# Autodesk Inventor assembly: ABD_Version_0.1_leftleg
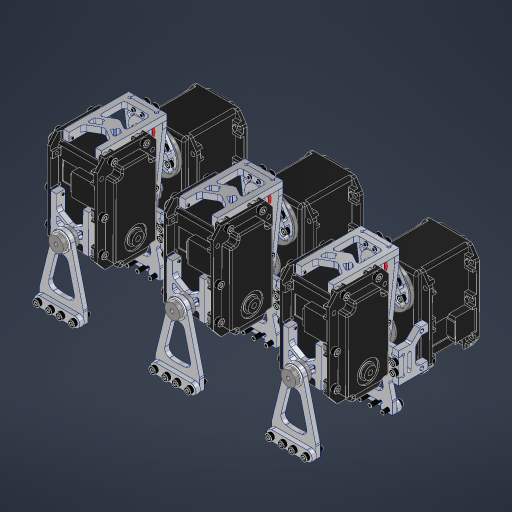
[picture p0: Inventor's stored thumbnail of the model, 512x512]
Saved by Autodesk Inventor 2024.3 (Build 283343000, 343)
## iProperties
Created: 2024-01-23
Part Number: ABD_Version_0.1_leftleg
Document SubType Name: Assembly
Designer: ASUS
Mass: 357.136 g
Surface Area: 604.848 cm^2
Volume: 181.423 cm^3
Density: 1.96853 g/cm^3
Author: ASUS
## Documents named in this file (26)
- C:\Users\ASUS\Desktop\Anti_Backlash_Structure_OP\v2_Frame\ABD_V2_Left_OP.iam
- C:\Users\ASUS\Desktop\ABD_2024_Eindhoven\MISUMI\Crank_Slider_Fixer.iam
- C:\Users\ASUS\Desktop\Anti_Backlash_Structure_OP\v2_Frame\Roll_Fixation_Set.iam
- C:\Users\ASUS\Desktop\Anti_Backlash_Structure_OP\v2_Frame\ABD_MX_64_Roll_Fixation_Set.iam
- C:\Users\ASUS\Desktop\Anti_Backlash_Structure_OP\v2_Frame\ABD_MX_64_Slider_Fixation_Set_Right2Horn.iam
- C:\Users\ASUS\Desktop\Anti_Backlash_Structure_OP\v2_Frame\ABD_Slider_Set_v2.iam
- C:\Users\ASUS\Desktop\Anti_Backlash_Structure_OP\v2_Frame\Roll_Fixation_Frame.ipt
- C:\Users\ASUS\Desktop\Anti_Backlash_Structure_OP\v2_Frame\Roll_Fixation_Frame_Back.ipt
- C:\Users\ASUS\Desktop\Anti_Backlash_Structure_OP\v2_Frame\hip joint fix washer.ipt
- C:\Users\ASUS\Desktop\ABD_2024_Eindhoven\MISUMI\hip_joint_fix_washer_10mm_Set.iam
- C:\Users\ASUS\Desktop\Anti_Backlash_Structure_OP\v2_Frame\Front_Frame_Fixer_v2.iam
- C:\Users\ASUS\Desktop\Anti_Backlash_Structure_OP\v2_Frame\Roll_Fixation_Frameto64.ipt
- C:\Users\ASUS\Desktop\ABD_2024_Eindhoven\MISUMI\CSH-ST-M2_5-6_203.ipt
- C:\Users\ASUS\Desktop\Anti_Backlash_Structure_OP\ROBOTIS(Inventor 2024 ver.)\DXL\MX-64T.ipt
- C:\Users\ASUS\Desktop\ABD_2024_Eindhoven\MISUMI\DBSY4-5-8.ipt
- C:\Users\ASUS\Desktop\ABD_2024_Eindhoven\MISUMI\C-WSSA12-4-2.ipt
- C:\Users\ASUS\Desktop\ABD_2024_Eindhoven\MISUMI\TT-0822-10.ipt
- C:\Users\ASUS\Desktop\ABD_2024_Eindhoven\MISUMI\CSHCS-SUSTBS-M4-20_214.ipt
- C:\Users\ASUS\Desktop\ABD_2024_Eindhoven\MISUMI\SLBNR4.ipt
- C:\Users\ASUS\Desktop\Anti_Backlash_Structure_OP\MISUMI\80F-0610.ipt
- C:\Users\ASUS\Desktop\ABD_2024_Eindhoven\MISUMI\C-WSSA12-8-3.ipt
- C:\Users\ASUS\Desktop\ABD_2024_Eindhoven\MISUMI\C-WSSA8-4-1.ipt
- C:\Users\ASUS\Desktop\Anti_Backlash_Structure_OP\V2_Frame(2025)\CSHBTT-ST-M4-18_203.ipt
- C:\Users\ASUS\Desktop\Anti_Backlash_Structure_OP\MISUMI\80F-0608.ipt
- C:\Users\ASUS\Desktop\ABD_2024_Eindhoven\MISUMI\E-GPWSSS12-4-1.ipt
- C:\Users\ASUS\Desktop\Anti_Backlash_Structure_OP\V2_Frame(2025)\M4-D6-9mm_Spacer.ipt
## Components (67 placed, 25 different names)
1. ABD_Slider_Set_v2:1 [sub-assembly]
2. Roll_Fixation_Set:1 [sub-assembly] — 삽입:5, 삽입:6, 각도:1, 플러쉬:4, 플러쉬:5, 플러쉬:7, 플러쉬:8, 메이트:43
3. Crank_Slider_Fixer:1 [sub-assembly] — 메이트:4
4. ABD_MX_64_Roll_Fixation_Set:1 [sub-assembly] — 메이트:2, 메이트:3, 삽입:5, 각도:1
5. ABD_MX_64_Slider_Fixation_Set_Right2Horn:1 [sub-assembly] — 메이트:2, 메이트:3, 삽입:6, 메이트:4
6. C-WSSA12-4-2:1 — 삽입:13, 삽입:15, 삽입:37
7. TT-0822-10:1 — 삽입:16, 삽입:36, 삽입:39
8. CSHCS-SUSTBS-M4-20_214:1
9. SLBNR4:1 — 삽입:13
10. 80F-0610:1 — 삽입:15, 삽입:16
11. Roll_Fixation_Frame:1
12. Roll_Fixation_Frame_Back:1 — 삽입:36
13. hip joint fix washer:1
14. hip joint fix washer:2
15. hip_joint_fix_washer_10mm_Set:1 [sub-assembly]
16. hip_joint_fix_washer_10mm_Set:2 [sub-assembly]
17. Front_Frame_Fixer_v2:1 [sub-assembly]
18. Roll_Fixation_Frameto64:1
19. Roll_Fixation_Frameto64:2
20. CSH-ST-M2_5-6_203:1
21. CSH-ST-M2_5-6_203:2
22. CSH-ST-M2_5-6_203:3
23. CSH-ST-M2_5-6_203:4
24. CSH-ST-M2_5-6_203:5
25. CSH-ST-M2_5-6_203:6
26. CSH-ST-M2_5-6_203:7
27. CSH-ST-M2_5-6_203:8
28. MX-64T:1 — 플러쉬:3, 메이트:26, 플러쉬:4, 플러쉬:5, 각도:2, 메이트:44
29. DBSY4-5-8:1
30. ABD_MX_64_Roll_Fixation_Set:2 [sub-assembly] — 삽입:37, 메이트:25, 각도:2
31. ABD_Slider_Set_v2:3 [sub-assembly] — 플러쉬:3, 메이트:26
32. Crank_Slider_Fixer:3 [sub-assembly]
33. ABD_MX_64_Slider_Fixation_Set_Right2Horn:3 [sub-assembly] — 삽입:39, 메이트:25, 삽입:40
34. C-WSSA12-8-3:1 — 삽입:40, 삽입:41
35. C-WSSA8-4-1:1 — 삽입:41, 삽입:42
36. CSHBTT-ST-M4-18_203:1 — 삽입:42
37. SLBNR4:2 — 삽입:83, 각도:4
38. Roll_Fixation_Frame:2
39. Roll_Fixation_Frame_Back:2 — 메이트:45
40. hip joint fix washer:3
41. hip joint fix washer:4
42. hip_joint_fix_washer_10mm_Set:3 [sub-assembly]
43. hip_joint_fix_washer_10mm_Set:4 [sub-assembly]
44. Front_Frame_Fixer_v2:2 [sub-assembly] — 삽입:85
45. Roll_Fixation_Frameto64:3
46. Roll_Fixation_Frameto64:4
47. CSH-ST-M2_5-6_203:9
48. CSH-ST-M2_5-6_203:10
49. CSH-ST-M2_5-6_203:11
50. CSH-ST-M2_5-6_203:12
51. CSH-ST-M2_5-6_203:13
52. CSH-ST-M2_5-6_203:14
53. CSH-ST-M2_5-6_203:15
54. CSH-ST-M2_5-6_203:16
55. MX-64T:2 — 플러쉬:7, 플러쉬:8, 메이트:43, 메이트:44
56. DBSY4-5-8:2
57. ABD_MX_64_Roll_Fixation_Set:3 [sub-assembly] — 삽입:82, 각도:4, 메이트:46, 삽입:85
58. ABD_Slider_Set_v2:4 [sub-assembly]
59. Crank_Slider_Fixer:4 [sub-assembly]
60. ABD_MX_64_Slider_Fixation_Set_Right2Horn:4 [sub-assembly] — 메이트:45, 메이트:46, 삽입:84
61. C-WSSA12-4-2:3 — 삽입:76, 삽입:82, 삽입:83
62. TT-0822-10:3 — 삽입:77, 삽입:78, 삽입:84
63. CSHBTT-ST-M4-18_203:3 — 삽입:79
64. 80F-0608:1 — 삽입:76, 삽입:77
65. TT-0822-10:4 — 삽입:78, 삽입:80
66. E-GPWSSS12-4-1:1 — 삽입:79, 삽입:81
67. M4-D6-9mm_Spacer:1 — 삽입:80, 삽입:81
## Relationships (111: Insert 63, Mate 38, Flush 6, Angle 4)
- [Insert]: ABD_Slider_Set_v2:1 ↔ Roll_Fixation_Set:1
- [Insert]: ABD_Slider_Set_v2:1 ↔ Crank_Slider_Fixer:1
- 메이트:2 [Mate] (0.05 mm): ABD_MX_64_Roll_Fixation_Set:1 ↔ ABD_MX_64_Slider_Fixation_Set_Right2Horn:1
- 메이트:3 [Mate]: ABD_MX_64_Roll_Fixation_Set:1 ↔ ABD_MX_64_Slider_Fixation_Set_Right2Horn:1
- 삽입:5 [Insert]: Roll_Fixation_Set:1 ↔ ABD_MX_64_Roll_Fixation_Set:1
- 삽입:6 [Insert]: Roll_Fixation_Set:1 ↔ ABD_MX_64_Slider_Fixation_Set_Right2Horn:1
- 메이트:4 [Mate]: Crank_Slider_Fixer:1 ↔ ABD_MX_64_Slider_Fixation_Set_Right2Horn:1
- 각도:1 [Angle] (0 deg): Roll_Fixation_Set:1 ↔ ABD_MX_64_Roll_Fixation_Set:1
- [Mate]: CSHCS-SUSTBS-M4-20_214:1 ↔ SLBNR4:1
- 삽입:13 [Insert] (1 mm): C-WSSA12-4-2:1 ↔ SLBNR4:1
- 삽입:15 [Insert]: C-WSSA12-4-2:1 ↔ 80F-0610:1
- 삽입:16 [Insert] (3 mm): TT-0822-10:1 ↔ 80F-0610:1
- [Mate]: Roll_Fixation_Frame:1 ↔ Roll_Fixation_Frame_Back:1
- [Insert]: Roll_Fixation_Frame:1 ↔ hip joint fix washer:1
- [Insert]: Roll_Fixation_Frame:1 ↔ hip joint fix washer:1
- [Insert]: Roll_Fixation_Frame_Back:1 ↔ hip joint fix washer:2
- [Mate]: Roll_Fixation_Frame_Back:1 ↔ hip joint fix washer:2
- [Mate]: Roll_Fixation_Frame_Back:1 ↔ hip joint fix washer:1
- [Mate]: Roll_Fixation_Frame_Back:1 ↔ hip joint fix washer:1
- [Mate]: Roll_Fixation_Frame:1 ↔ hip joint fix washer:1
- [Insert]: hip joint fix washer:1 ↔ hip_joint_fix_washer_10mm_Set:1
- [Mate]: hip joint fix washer:1 ↔ hip_joint_fix_washer_10mm_Set:1
- [Insert]: hip joint fix washer:2 ↔ hip_joint_fix_washer_10mm_Set:2
- [Mate]: hip joint fix washer:2 ↔ hip_joint_fix_washer_10mm_Set:2
- [Mate] (49 mm): Roll_Fixation_Frame:1 ↔ Roll_Fixation_Frame_Back:1
- [Mate]: hip_joint_fix_washer_10mm_Set:1 ↔ hip_joint_fix_washer_10mm_Set:2
- [Mate]: hip_joint_fix_washer_10mm_Set:1 ↔ hip_joint_fix_washer_10mm_Set:2
- [Insert]: Roll_Fixation_Frame_Back:1 ↔ Roll_Fixation_Frameto64:2
- [Insert]: Roll_Fixation_Frame_Back:1 ↔ Roll_Fixation_Frameto64:1
- [Mate]: Roll_Fixation_Frame_Back:1 ↔ Roll_Fixation_Frameto64:2
- [Mate]: Roll_Fixation_Frame_Back:1 ↔ Roll_Fixation_Frameto64:1
- [Insert]: Roll_Fixation_Frame_Back:1 ↔ CSH-ST-M2_5-6_203:2
- [Insert]: Roll_Fixation_Frame_Back:1 ↔ CSH-ST-M2_5-6_203:1
- [Insert]: Roll_Fixation_Frame_Back:1 ↔ CSH-ST-M2_5-6_203:3
- [Insert]: Roll_Fixation_Frame_Back:1 ↔ CSH-ST-M2_5-6_203:4
- [Insert] (2.5 mm): Roll_Fixation_Frameto64:2 ↔ CSH-ST-M2_5-6_203:7
- [Insert] (2.5 mm): Roll_Fixation_Frameto64:1 ↔ CSH-ST-M2_5-6_203:6
- [Insert] (2.5 mm): Roll_Fixation_Frameto64:1 ↔ CSH-ST-M2_5-6_203:5
- [Insert] (2.5 mm): Roll_Fixation_Frameto64:2 ↔ CSH-ST-M2_5-6_203:8
- [Insert]: Roll_Fixation_Frameto64:1 ↔ MX-64T:1
- [Insert]: Roll_Fixation_Frameto64:1 ↔ MX-64T:1
- [Insert]: Front_Frame_Fixer_v2:1 ↔ DBSY4-5-8:1
- [Insert]: Roll_Fixation_Frame:1 ↔ Front_Frame_Fixer_v2:1
- 삽입:36 [Insert]: TT-0822-10:1 ↔ Roll_Fixation_Frame_Back:1
- 삽입:37 [Insert]: C-WSSA12-4-2:1 ↔ ABD_MX_64_Roll_Fixation_Set:2
- [Insert]: ABD_Slider_Set_v2:3 ↔ Crank_Slider_Fixer:3
- [Mate]: Crank_Slider_Fixer:3 ↔ ABD_MX_64_Slider_Fixation_Set_Right2Horn:3
- 삽입:39 [Insert]: TT-0822-10:1 ↔ ABD_MX_64_Slider_Fixation_Set_Right2Horn:3
- 메이트:25 [Mate]: ABD_MX_64_Roll_Fixation_Set:2 ↔ ABD_MX_64_Slider_Fixation_Set_Right2Horn:3
- 플러쉬:3 [Flush] (-3 mm): MX-64T:1 ↔ ABD_Slider_Set_v2:3
- 메이트:26 [Mate]: MX-64T:1 ↔ ABD_Slider_Set_v2:3
- 플러쉬:4 [Flush]: Roll_Fixation_Set:1 ↔ MX-64T:1
- 플러쉬:5 [Flush]: Roll_Fixation_Set:1 ↔ MX-64T:1
- 삽입:40 [Insert]: ABD_MX_64_Slider_Fixation_Set_Right2Horn:3 ↔ C-WSSA12-8-3:1
- 삽입:41 [Insert]: C-WSSA12-8-3:1 ↔ C-WSSA8-4-1:1
- 삽입:42 [Insert]: C-WSSA8-4-1:1 ↔ CSHBTT-ST-M4-18_203:1
- 각도:2 [Angle] (0 deg): MX-64T:1 ↔ ABD_MX_64_Roll_Fixation_Set:2
- [Mate]: Roll_Fixation_Frame:2 ↔ Roll_Fixation_Frame_Back:2
- [Insert]: Roll_Fixation_Frame:2 ↔ hip joint fix washer:3
- [Insert]: Roll_Fixation_Frame:2 ↔ hip joint fix washer:3
- [Insert]: Roll_Fixation_Frame_Back:2 ↔ hip joint fix washer:4
- [Mate]: Roll_Fixation_Frame_Back:2 ↔ hip joint fix washer:4
- [Mate]: Roll_Fixation_Frame_Back:2 ↔ hip joint fix washer:3
- [Mate]: Roll_Fixation_Frame_Back:2 ↔ hip joint fix washer:3
- [Mate]: Roll_Fixation_Frame:2 ↔ hip joint fix washer:3
- [Insert]: hip joint fix washer:3 ↔ hip_joint_fix_washer_10mm_Set:3
- [Mate]: hip joint fix washer:3 ↔ hip_joint_fix_washer_10mm_Set:3
- [Insert]: hip joint fix washer:4 ↔ hip_joint_fix_washer_10mm_Set:4
- [Mate]: hip joint fix washer:4 ↔ hip_joint_fix_washer_10mm_Set:4
- [Mate] (49 mm): Roll_Fixation_Frame:2 ↔ Roll_Fixation_Frame_Back:2
- [Mate]: hip_joint_fix_washer_10mm_Set:3 ↔ hip_joint_fix_washer_10mm_Set:4
- [Mate]: hip_joint_fix_washer_10mm_Set:3 ↔ hip_joint_fix_washer_10mm_Set:4
- [Insert]: Roll_Fixation_Frame_Back:2 ↔ Roll_Fixation_Frameto64:4
- [Insert]: Roll_Fixation_Frame_Back:2 ↔ Roll_Fixation_Frameto64:3
- [Mate]: Roll_Fixation_Frame_Back:2 ↔ Roll_Fixation_Frameto64:4
- [Mate]: Roll_Fixation_Frame_Back:2 ↔ Roll_Fixation_Frameto64:3
- [Insert]: Roll_Fixation_Frame_Back:2 ↔ CSH-ST-M2_5-6_203:10
- [Insert]: Roll_Fixation_Frame_Back:2 ↔ CSH-ST-M2_5-6_203:9
- [Insert]: Roll_Fixation_Frame_Back:2 ↔ CSH-ST-M2_5-6_203:11
- [Insert]: Roll_Fixation_Frame_Back:2 ↔ CSH-ST-M2_5-6_203:12
- [Insert] (2.5 mm): Roll_Fixation_Frameto64:4 ↔ CSH-ST-M2_5-6_203:15
- [Insert] (2.5 mm): Roll_Fixation_Frameto64:3 ↔ CSH-ST-M2_5-6_203:14
- [Insert] (2.5 mm): Roll_Fixation_Frameto64:3 ↔ CSH-ST-M2_5-6_203:13
- [Insert] (2.5 mm): Roll_Fixation_Frameto64:4 ↔ CSH-ST-M2_5-6_203:16
- [Insert]: Roll_Fixation_Frameto64:3 ↔ MX-64T:2
- [Insert]: Roll_Fixation_Frameto64:3 ↔ MX-64T:2
- [Insert]: Front_Frame_Fixer_v2:2 ↔ DBSY4-5-8:2
- [Insert]: Roll_Fixation_Frame:2 ↔ Front_Frame_Fixer_v2:2
- [Insert]: ABD_Slider_Set_v2:4 ↔ Crank_Slider_Fixer:4
- [Mate]: Crank_Slider_Fixer:4 ↔ ABD_MX_64_Slider_Fixation_Set_Right2Horn:4
- [Mate]: ABD_MX_64_Roll_Fixation_Set:3 ↔ ABD_MX_64_Slider_Fixation_Set_Right2Horn:4
- [Flush] (-3 mm): MX-64T:2 ↔ ABD_Slider_Set_v2:4
- [Mate]: MX-64T:2 ↔ ABD_Slider_Set_v2:4
- [Angle] (0 deg): MX-64T:2 ↔ ABD_MX_64_Roll_Fixation_Set:3
- 플러쉬:7 [Flush]: Roll_Fixation_Set:1 ↔ MX-64T:2
- 플러쉬:8 [Flush]: Roll_Fixation_Set:1 ↔ MX-64T:2
- 메이트:43 [Mate] (50 mm): Roll_Fixation_Set:1 ↔ MX-64T:2
- 메이트:44 [Mate] (50 mm): MX-64T:1 ↔ MX-64T:2
- 삽입:76 [Insert]: C-WSSA12-4-2:3 ↔ 80F-0608:1
- 삽입:77 [Insert] (3 mm): TT-0822-10:3 ↔ 80F-0608:1
- 삽입:78 [Insert] (3 mm): TT-0822-10:3 ↔ TT-0822-10:4
- 삽입:79 [Insert]: CSHBTT-ST-M4-18_203:3 ↔ E-GPWSSS12-4-1:1
- 삽입:80 [Insert]: TT-0822-10:4 ↔ M4-D6-9mm_Spacer:1
- 삽입:81 [Insert]: E-GPWSSS12-4-1:1 ↔ M4-D6-9mm_Spacer:1
- 메이트:45 [Mate]: Roll_Fixation_Frame_Back:2 ↔ ABD_MX_64_Slider_Fixation_Set_Right2Horn:4
- 삽입:82 [Insert]: ABD_MX_64_Roll_Fixation_Set:3 ↔ C-WSSA12-4-2:3
- 삽입:83 [Insert] (1 mm): SLBNR4:2 ↔ C-WSSA12-4-2:3
- 각도:4 [Angle] (0 deg): SLBNR4:2 ↔ ABD_MX_64_Roll_Fixation_Set:3
- 메이트:46 [Mate]: ABD_MX_64_Roll_Fixation_Set:3 ↔ ABD_MX_64_Slider_Fixation_Set_Right2Horn:4
- 삽입:84 [Insert]: ABD_MX_64_Slider_Fixation_Set_Right2Horn:4 ↔ TT-0822-10:3
- 삽입:85 [Insert]: Front_Frame_Fixer_v2:2 ↔ ABD_MX_64_Roll_Fixation_Set:3
## Named parameters: d1045_d987_d190 = 0 mm, d1046_d992_d946 = 0 mm, d1061_d1045_d987_d190 = 0 mm, d1062_d1046_d992_d946 = 0 mm, d1064_d1048 = 0 mm, d1065_d1049 = -3 mm, d1066_d1050 = 0 mm, d1072_d1058 = 0 deg, d1075_d838 = 0 mm, d1076_d839 = 0 mm, d1077_d840 = 0 mm, d1078_d841 = 0 mm, d1079_d587 = 0 mm, d1080_d753 = 0 mm, d1081_d754 = 0 mm, d1082_d756 = 0 mm, d1083_d757 = 0 mm, d1084_d761 = 0 mm, d1085_d762 = 0 mm, d1086_d764 = 0 mm, d1087_d49 = 0 mm, d1088_d50 = 0 mm, d1089_d16 = 49 mm, d1090_d17 = 0 mm, d1091_d18 = 0 mm, d1092_d20 = 0 mm, d1093_d21 = 0 mm, d1094_d22 = 0 mm, d1095_d23 = 0 mm, d1096_d24 = 0 mm, d1097_d25 = 0 mm, d1098_d26 = 0 mm, d1099_d27 = 0 mm, d1100_d31 = 2.5 mm, d1101_d32 = 2.5 mm, d1102_d33 = 2.5 mm, d1103_d34 = 2.5 mm, d1104_d35 = 0 mm, d1105_d36 = 0 mm
